# Autodesk Inventor assembly: 000.200 - Средняя ось
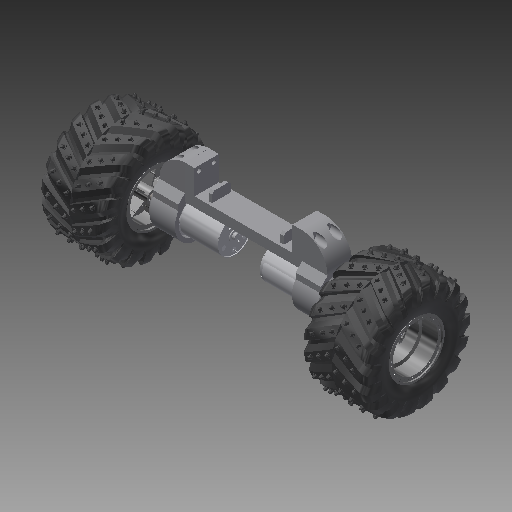
[picture p0: Inventor's stored thumbnail of the model, 512x512]
Saved by Autodesk Inventor 2019 (Build 230136000, 136)
## iProperties
Created: 2020-06-06
Part Number: 000.200 - Средняя ось
Material: Типовые
Document SubType Name: Assembly
Designer: Петров Иван
Author: Петров Иван
## Documents named in this file (5)
- E:\IVAN\Ivan_desktop\My_projects\RTK\000.200 - Средняя ось.iam
- E:\IVAN\Ivan_desktop\My_projects\RTK\000.201 - Балка несущая.ipt
- E:\IVAN\Ivan_desktop\My_projects\RTK\000.202 - Кожух мотора.ipt
- E:\IVAN\Ivan_desktop\My_projects\RTK\components\39530_txm-dc gearhead motor.ipt
- E:\IVAN\Ivan_desktop\My_projects\RTK\components\Колесо\Wheel1.iam
## Components (7 placed, 4 different names)
1. 000.201 - Балка несущая:1 — Совмещение:7, Совмещение:8, Касательность:1, Касательность:2, Совмещение:9, Совмещение:10, Совмещение:11
2. 000.202 - Кожух мотора:1 — Совмещение:2, Совмещение:3, Совмещение:4, Совмещение:7, Совмещение:9, Совмещение:10
3. 39530_txm-dc gearhead motor:1 — Совмещение:1, Совмещение:5, Совмещение:6, Касательность:1, Совмещение:14, Совмещение:15
4. 39530_txm-dc gearhead motor:2 — Совмещение:2, Совмещение:3, Совмещение:4, Касательность:2, Совмещение:12, Совмещение:13
5. 000.202 - Кожух мотора:2 — Совмещение:1, Совмещение:5, Совмещение:6, Совмещение:8, Совмещение:11
6. Wheel1:1 [sub-assembly] — Совмещение:12, Совмещение:13
7. Wheel1:2 [sub-assembly] — Совмещение:14, Совмещение:15
## Relationships (17: Mate 15, Tangent 2)
- Совмещение:1 [Mate]: 39530_txm-dc gearhead motor:1 ↔ 000.202 - Кожух мотора:2
- Совмещение:2 [Mate]: 000.202 - Кожух мотора:1 ↔ 39530_txm-dc gearhead motor:2
- Совмещение:3 [Mate]: 000.202 - Кожух мотора:1 ↔ 39530_txm-dc gearhead motor:2
- Совмещение:4 [Mate]: 000.202 - Кожух мотора:1 ↔ 39530_txm-dc gearhead motor:2
- Совмещение:5 [Mate]: 39530_txm-dc gearhead motor:1 ↔ 000.202 - Кожух мотора:2
- Совмещение:6 [Mate]: 39530_txm-dc gearhead motor:1 ↔ 000.202 - Кожух мотора:2
- Совмещение:7 [Mate]: 000.201 - Балка несущая:1 ↔ 000.202 - Кожух мотора:1
- Совмещение:8 [Mate]: 000.201 - Балка несущая:1 ↔ 000.202 - Кожух мотора:2
- Касательность:1 [Tangent]: 000.201 - Балка несущая:1 ↔ 39530_txm-dc gearhead motor:1
- Касательность:2 [Tangent]: 000.201 - Балка несущая:1 ↔ 39530_txm-dc gearhead motor:2
- Совмещение:9 [Mate]: 000.201 - Балка несущая:1 ↔ 000.202 - Кожух мотора:1
- Совмещение:10 [Mate]: 000.201 - Балка несущая:1 ↔ 000.202 - Кожух мотора:1
- Совмещение:11 [Mate]: 000.201 - Балка несущая:1 ↔ 000.202 - Кожух мотора:2
- Совмещение:12 [Mate]: 39530_txm-dc gearhead motor:2 ↔ Wheel1:1
- Совмещение:13 [Mate]: 39530_txm-dc gearhead motor:2 ↔ Wheel1:1
- Совмещение:14 [Mate]: 39530_txm-dc gearhead motor:1 ↔ Wheel1:2
- Совмещение:15 [Mate]: 39530_txm-dc gearhead motor:1 ↔ Wheel1:2
